# Autodesk Inventor assembly: box assembly
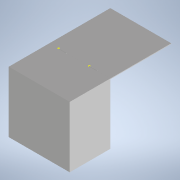
[picture p0: Inventor's stored thumbnail of the model, 180x180]
Saved by Autodesk Inventor 2021 (Build 250183000, 183)
## iProperties
Created: 2023-06-03
Part Number: box assembly
Document SubType Name: Assembly
Designer: Sahil Nadaf
Author: Sahil Nadaf
## Documents named in this file (4)
- D:\Engg exploration\box assembly.iam
- D:\Engg exploration\rectangle box.ipt
- D:\Engg exploration\middle portion.ipt
- D:\Engg exploration\rectangle upper portion.ipt
## Components (4 placed, 3 different names)
1. rectangle box:1 — Rigid:1, Rigid:2, Rotational:1
2. middle portion:1 — Rigid:2
3. middle portion:2 — Rigid:1
4. rectangle upper portion:1 — Rotational:1
## Relationships (3: WeldJoint 2, RevoluteJoint 1)
- Rigid:1 [WeldJoint] (-100 mm): rectangle box:1 ↔ middle portion:2
- Rigid:2 [WeldJoint] (-100 mm): rectangle box:1 ↔ middle portion:1
- Rotational:1 [RevoluteJoint]: rectangle box:1 ↔ rectangle upper portion:1
